# Autodesk Inventor assembly: Assembly
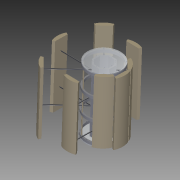
[picture p0: Inventor's stored thumbnail of the model, 180x180]
Saved by Autodesk Inventor 2015 (Build 190159000, 159)
## iProperties
Created: 2015-09-23
Part Number: Assembly
Document SubType Name: Assembly
Designer: Stefania
Author: Stefania
## Documents named in this file (8)
- C:\Users\Stefania\SkyDrive\Documents\ME102B\Inventor\ActualDesigns\Assembly.iam
- C:\Users\Stefania\SkyDrive\Documents\ME102B\Inventor\ActualDesigns\Part1.ipt
- C:\Users\Stefania\SkyDrive\Documents\ME102B\Inventor\ActualDesigns\LongitudinalSupportBar.ipt
- C:\Users\Stefania\SkyDrive\Documents\ME102B\Inventor\ActualDesigns\EndCap.ipt
- C:\Users\Stefania\SkyDrive\Documents\ME102B\Inventor\ActualDesigns\CentralRod_v1.2.ipt
- C:\Users\Stefania\SkyDrive\Documents\ME102B\Inventor\ActualDesigns\LeadScrew.ipt
- C:\Users\Stefania\SkyDrive\Documents\ME102B\Inventor\ActualDesigns\Foot1.ipt
- C:\Users\Stefania\SkyDrive\Documents\ME102B\Inventor\ActualDesigns\Foot2.ipt
## Components (28 placed, 7 different names)
1. Part1:1 — Rigid:1, Rigid:2, Rigid:3, Rigid:4, Rigid:5, Rigid:6, Rigid:7, Rigid:8, Rigid:9, Rigid:10
2. LongitudinalSupportBar:1 — Rigid:8
3. LongitudinalSupportBar:2 — Rigid:7
4. LongitudinalSupportBar:3 — Rigid:6
5. LongitudinalSupportBar:4 — Rigid:5
6. LongitudinalSupportBar:5 — Rigid:4
7. LongitudinalSupportBar:6 — Rigid:3
8. LongitudinalSupportBar:7 — Rigid:2
9. LongitudinalSupportBar:8 — Rigid:1
10. EndCap:1 — Rigid:9
11. EndCap:2 — Rigid:10, Rigid:11
12. CentralRod_v1.2:1 — Rigid:11, Cylindrical:1, Cylindrical:3, Cylindrical:4, Cylindrical:5, Cylindrical:6, Cylindrical:7, Cylindrical:8, Cylindrical:9
13. LeadScrew:1 — Cylindrical:9, Flush:6, Mate:9, Rigid:16, Mate:11
14. LeadScrew:2 — Cylindrical:1, Flush:5, Mate:5, Rigid:14, Mate:7, Rigid:15
15. LeadScrew:3 — Cylindrical:4, Flush:6, Mate:10, Mate:12, Rigid:17
16. LeadScrew:4 — Cylindrical:5, Flush:2, Mate:1, Mate:4
17. LeadScrew:5 — Cylindrical:3, Flush:5, Mate:6, Mate:8
18. LeadScrew:6 — Cylindrical:6, Flush:3, Flush:4, Mate:14, Rigid:18, Mate:15
19. LeadScrew:7 — Cylindrical:7, Flush:2, Mate:2, Rigid:12, Mate:3, Rigid:13
20. LeadScrew:8 — Cylindrical:8, Flush:3, Flush:4, Mate:13, Mate:16, Rigid:19
21. Foot1:1 — Mate:3, Mate:4, Rigid:13
22. Foot1:2 — Mate:1, Mate:2, Rigid:12
23. Foot2:1 — Mate:5, Mate:6, Rigid:14
24. Foot2:2 — Mate:7, Mate:8, Rigid:15
25. Foot1:3 — Mate:9, Mate:10, Rigid:16
26. Foot1:4 — Mate:11, Mate:12, Rigid:17
27. Foot2:3 — Mate:13, Mate:14, Rigid:18
28. Foot2:4 — Mate:15, Mate:16, Rigid:19
## Relationships (48: WeldJoint 19, Mate 16, CylindricalJoint 8, Flush 5)
- Rigid:1 [WeldJoint]: Part1:1 ↔ LongitudinalSupportBar:8
- Rigid:2 [WeldJoint]: Part1:1 ↔ LongitudinalSupportBar:7
- Rigid:3 [WeldJoint]: Part1:1 ↔ LongitudinalSupportBar:6
- Rigid:4 [WeldJoint]: Part1:1 ↔ LongitudinalSupportBar:5
- Rigid:5 [WeldJoint]: Part1:1 ↔ LongitudinalSupportBar:4
- Rigid:6 [WeldJoint]: Part1:1 ↔ LongitudinalSupportBar:3
- Rigid:7 [WeldJoint]: Part1:1 ↔ LongitudinalSupportBar:2
- Rigid:8 [WeldJoint]: Part1:1 ↔ LongitudinalSupportBar:1
- Rigid:9 [WeldJoint]: Part1:1 ↔ EndCap:1
- Rigid:10 [WeldJoint]: Part1:1 ↔ EndCap:2
- Rigid:11 [WeldJoint]: EndCap:2 ↔ CentralRod_v1.2:1
- Cylindrical:1: CentralRod_v1.2:1 ↔ LeadScrew:2
- Cylindrical:3: CentralRod_v1.2:1 ↔ LeadScrew:5
- Cylindrical:4: CentralRod_v1.2:1 ↔ LeadScrew:3
- Cylindrical:5: CentralRod_v1.2:1 ↔ LeadScrew:4
- Cylindrical:6: CentralRod_v1.2:1 ↔ LeadScrew:6
- Cylindrical:7: CentralRod_v1.2:1 ↔ LeadScrew:7
- Cylindrical:8: CentralRod_v1.2:1 ↔ LeadScrew:8
- Cylindrical:9: CentralRod_v1.2:1 ↔ LeadScrew:1
- Flush:2: LeadScrew:4 ↔ LeadScrew:7
- Flush:3: LeadScrew:6 ↔ LeadScrew:8
- Flush:4: LeadScrew:6 ↔ LeadScrew:8
- Flush:5: LeadScrew:2 ↔ LeadScrew:5
- Flush:6: LeadScrew:1 ↔ LeadScrew:3
- Mate:1: LeadScrew:4 ↔ Foot1:2
- Mate:2: LeadScrew:7 ↔ Foot1:2
- Rigid:12 [WeldJoint]: LeadScrew:7 ↔ Foot1:2
- Mate:3: LeadScrew:7 ↔ Foot1:1
- Mate:4: LeadScrew:4 ↔ Foot1:1
- Rigid:13 [WeldJoint]: LeadScrew:7 ↔ Foot1:1
- Mate:5: LeadScrew:2 ↔ Foot2:1
- Mate:6: LeadScrew:5 ↔ Foot2:1
- Rigid:14 [WeldJoint]: LeadScrew:2 ↔ Foot2:1
- Mate:7: LeadScrew:2 ↔ Foot2:2
- Mate:8: LeadScrew:5 ↔ Foot2:2
- Rigid:15 [WeldJoint]: LeadScrew:2 ↔ Foot2:2
- Mate:9: LeadScrew:1 ↔ Foot1:3
- Mate:10: LeadScrew:3 ↔ Foot1:3
- Rigid:16 [WeldJoint]: LeadScrew:1 ↔ Foot1:3
- Mate:11: LeadScrew:1 ↔ Foot1:4
- Mate:12: LeadScrew:3 ↔ Foot1:4
- Rigid:17 [WeldJoint]: LeadScrew:3 ↔ Foot1:4
- Mate:13: LeadScrew:8 ↔ Foot2:3
- Mate:14: LeadScrew:6 ↔ Foot2:3
- Rigid:18 [WeldJoint]: LeadScrew:6 ↔ Foot2:3
- Mate:15: LeadScrew:6 ↔ Foot2:4
- Mate:16: LeadScrew:8 ↔ Foot2:4
- Rigid:19 [WeldJoint]: LeadScrew:8 ↔ Foot2:4
